# Autodesk Inventor assembly: GAMEMECH_FORKLIFT
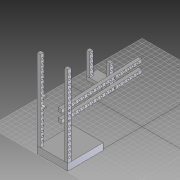
[picture p0: Inventor's stored thumbnail of the model, 180x180]
Saved by Autodesk Inventor 2015 (Build 190159000, 159)
## iProperties
Created: 2015-01-15
Part Number: GAMEMECH_FORKLIFT
Document SubType Name: Assembly
Designer: Tucker
Author: Tucker
## Documents named in this file (6)
- C:\Users\Tucker\Documents\GitHub\frc2015\CAD\GAMEMECH_FORKLIFT.iam
- C:\Users\Tucker\Documents\GitHub\frc2015\CAD\chasse.ipt
- C:\Users\Tucker\Documents\GitHub\frc2015\CAD\pole.ipt
- C:\Users\Tucker\Documents\GitHub\frc2015\CAD\box_forklift.ipt
- C:\Users\Tucker\Documents\GitHub\frc2015\CAD\axle_word_used_loosely.ipt
- C:\Users\Tucker\Documents\GitHub\frc2015\CAD\gripper_mc_dipper.ipt
## Components (14 placed, 5 different names)
1. chasse:1 — Mate:1, Flush:1, Flush:2, Mate:2, Flush:3, Flush:4
2. pole:1 — Mate:1, Flush:1, Flush:2, Mate:3, Rotation:1, Mate:4, Mate:6, Mate:7, Flush:6
3. pole:2 — Mate:2, Flush:3, Flush:4, Mate:5, Mate:8, Flush:5, Flush:7
4. box_forklift:1 — Mate:13, Flush:8, Flush:9, Mate:14, Flush:10, Flush:11
5. axle_word_used_loosely:1 — Mate:3, Rotation:1, Mate:4, Flush:6, Mate:9, Mate:10
6. axle_word_used_loosely:2 — Mate:6, Mate:7, Mate:11, Mate:12
7. axle_word_used_loosely:3 — Mate:5, Flush:7
8. axle_word_used_loosely:4 — Mate:8, Flush:5
9. pole:4 — Mate:9, Mate:10, Flush:16, Mate:21, Flush:17, Flush:20
10. pole:5 — Mate:11, Mate:12, Flush:16, Mate:22, Flush:18, Flush:19
11. gripper_mc_dipper:1 — Mate:13, Flush:8, Flush:9, Mate:19, Mate:20
12. gripper_mc_dipper:2 — Mate:14, Flush:10, Flush:11
13. axle_word_used_loosely:5 — Mate:20, Mate:22, Flush:18, Flush:19
14. axle_word_used_loosely:6 — Mate:19, Mate:21, Flush:17, Flush:20
## Relationships (35: Mate 18, Flush 16, RelateRotation 1)
- Mate:1: chasse:1 ↔ pole:1
- Flush:1: chasse:1 ↔ pole:1
- Flush:2: chasse:1 ↔ pole:1
- Mate:2: chasse:1 ↔ pole:2
- Flush:3: chasse:1 ↔ pole:2
- Flush:4: chasse:1 ↔ pole:2
- Mate:3: pole:1 ↔ axle_word_used_loosely:1
- Rotation:1 [RelateRotation] (1 ul): pole:1 ↔ axle_word_used_loosely:1
- Mate:4: pole:1 ↔ axle_word_used_loosely:1
- Mate:5: pole:2 ↔ axle_word_used_loosely:3
- Mate:6: pole:1 ↔ axle_word_used_loosely:2
- Mate:7: pole:1 ↔ axle_word_used_loosely:2
- Mate:8: pole:2 ↔ axle_word_used_loosely:4
- Flush:5: pole:2 ↔ axle_word_used_loosely:4
- Flush:6: pole:1 ↔ axle_word_used_loosely:1
- Flush:7: pole:2 ↔ axle_word_used_loosely:3
- Mate:9: axle_word_used_loosely:1 ↔ pole:4
- Mate:10: axle_word_used_loosely:1 ↔ pole:4
- Mate:11: axle_word_used_loosely:2 ↔ pole:5
- Mate:12: axle_word_used_loosely:2 ↔ pole:5
- Mate:13: box_forklift:1 ↔ gripper_mc_dipper:1
- Flush:8: box_forklift:1 ↔ gripper_mc_dipper:1
- Flush:9: box_forklift:1 ↔ gripper_mc_dipper:1
- Mate:14: box_forklift:1 ↔ gripper_mc_dipper:2
- Flush:10: box_forklift:1 ↔ gripper_mc_dipper:2
- Flush:11: box_forklift:1 ↔ gripper_mc_dipper:2
- Flush:16: pole:4 ↔ pole:5
- Mate:19: gripper_mc_dipper:1 ↔ axle_word_used_loosely:6
- Mate:20: gripper_mc_dipper:1 ↔ axle_word_used_loosely:5
- Mate:21: pole:4 ↔ axle_word_used_loosely:6
- Mate:22: pole:5 ↔ axle_word_used_loosely:5
- Flush:17: pole:4 ↔ axle_word_used_loosely:6
- Flush:18: pole:5 ↔ axle_word_used_loosely:5
- Flush:19: pole:5 ↔ axle_word_used_loosely:5
- Flush:20: pole:4 ↔ axle_word_used_loosely:6
